# Autodesk Inventor assembly: body
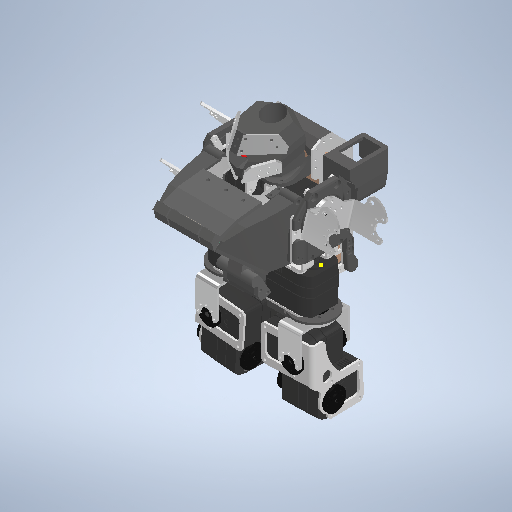
[picture p0: Inventor's stored thumbnail of the model, 512x512]
Saved by Autodesk Inventor 2026.1 (Build 301233020, 233B)
## iProperties
Created: 2024-10-10
Part Number: body
Document SubType Name: Assembly
Designer: hibik
Author: hibik
## Documents named in this file (7)
- C:\Users\hibik\Documents\Robomech\HR\Eglantyne_mark2\hard\body.iam
- C:\Users\hibik\Documents\Robomech\HR\Eglantyne_mark2\hard\under_body\under_body.iam
- C:\Users\hibik\Documents\Robomech\HR\Eglantyne_mark2\hard\needed_model\battely.ipt
- C:\Users\hibik\Documents\Robomech\HR\Eglantyne_mark2\hard\head\head.iam
- C:\Users\hibik\Documents\Robomech\HR\Eglantyne_mark2\hard\board\board.iam
- C:\Users\hibik\Documents\Robomech\HR\Eglantyne_mark2\hard\upper_body\upperbody.iam
- C:\Users\hibik\Documents\Robomech\HR\Eglantyne_mark2\hard\upper_body\chest\chest_cover.iam
## Components (6 placed, 6 different names)
1. under_body:1 [sub-assembly] — 挿入:1, 挿入:2, 角度:1
2. battely:1
3. board:1 [sub-assembly] — 挿入:1, 角度:3
4. upperbody:1 [sub-assembly] — 挿入:2, 角度:1, 挿入:3, 挿入:4, 角度:2, 角度:3
5. head:4 [sub-assembly] — 挿入:3
6. chest_cover:2 [sub-assembly] — 挿入:4, 角度:2
## Relationships (7: Insert 4, Angle 3)
- 挿入:1 [Insert] (0.5 mm): under_body:1 ↔ board:1
- 挿入:2 [Insert]: under_body:1 ↔ upperbody:1
- 角度:1 [Angle] (0 deg): under_body:1 ↔ upperbody:1
- 挿入:3 [Insert]: upperbody:1 ↔ head:4
- 挿入:4 [Insert] (0.5 mm): upperbody:1 ↔ chest_cover:2
- 角度:2 [Angle] (0 deg): upperbody:1 ↔ chest_cover:2
- 角度:3 [Angle] (0 deg): board:1 ↔ upperbody:1
